# Autodesk Inventor assembly: drill back cavity to neck pickup cavity hole
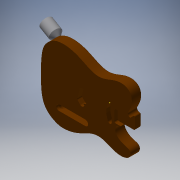
[picture p0: Inventor's stored thumbnail of the model, 180x180]
Saved by Autodesk Inventor 2018 (Build 220112000, 112)
## iProperties
Created: 2021-03-25
Part Number: drill back cavity to neck pickup cavity hole
Document SubType Name: Assembly
Designer: Charles.Rymal
Author: Charles.Rymal
## Documents named in this file (3)
- C:\Users\Charles.Rymal\source\guitar\CAD\drill back cavity to neck pickup cavity hole.iam
- C:\Users\Charles.Rymal\source\guitar\CAD\Body.ipt
- C:\Users\Charles.Rymal\source\guitar\CAD\Drill 12.ipt
## Components (2 placed, 2 different names)
1. Body:1 — Mate:1, Mate:2
2. Drill 12:1 — Mate:1, Mate:2
## Relationships (2: Mate 2)
- Mate:1: Body:1 ↔ Drill 12:1
- Mate:2: Body:1 ↔ Drill 12:1
